# Autodesk Inventor assembly: battery_lib_assy
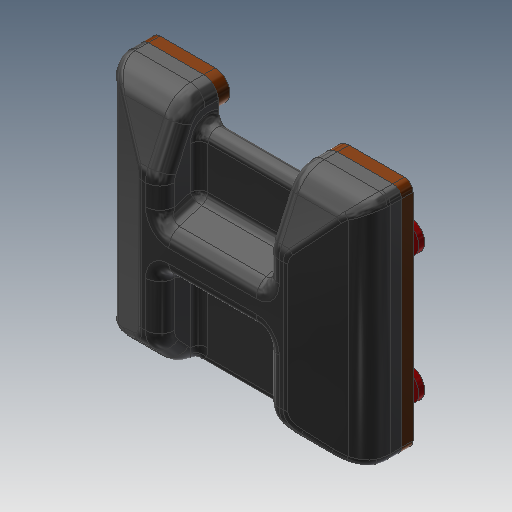
[picture p0: Inventor's stored thumbnail of the model, 512x512]
Saved by Autodesk Inventor 2019.4 (Build 234330000, 330)
## iProperties
Created: 2018-09-07
Part Number: battery_lib_assy
Material: 一般
Document SubType Name: Assembly
Designer: y6tada
Author: y6tada
## Documents named in this file (4)
- C:\Workspace\Yunit8-HaptHexa\Hardware\Inventor\Thorax\battery_lib_assy.iam
- C:\Workspace\Yunit8-HaptHexa\Hardware\Inventor\Thorax\battery_lid_print.ipt
- C:\Workspace\Yunit8-HaptHexa\Hardware\Inventor\Thorax\battery_cover_base.ipt
- C:\Workspace\Yunit8-HaptHexa\Hardware\Inventor\Thorax\battery_lib_hook.ipt
## Components (3 placed, 3 different names)
1. battery_cover_base:1 — メイト:1, フラッシュ:1, メイト:2, メイト:3, フラッシュ:2, メイト:4, フラッシュ:3, フラッシュ:5
2. battery_lid_print:1 — メイト:3, フラッシュ:2, メイト:4
3. battery_lib_hook:1 — フラッシュ:3, メイト:5, フラッシュ:4, フラッシュ:5
## Relationships (10: Mate 5, Flush 5)
- メイト:1 [Mate]: battery_cover_base:1
- フラッシュ:1 [Flush]: battery_cover_base:1
- メイト:2 [Mate]: battery_cover_base:1
- メイト:3 [Mate]: battery_cover_base:1 ↔ battery_lid_print:1
- フラッシュ:2 [Flush]: battery_cover_base:1 ↔ battery_lid_print:1
- メイト:4 [Mate]: battery_cover_base:1 ↔ battery_lid_print:1
- フラッシュ:3 [Flush]: battery_cover_base:1 ↔ battery_lib_hook:1
- メイト:5 [Mate]: battery_lib_hook:1
- フラッシュ:4 [Flush]: battery_lib_hook:1
- フラッシュ:5 [Flush]: battery_cover_base:1 ↔ battery_lib_hook:1
